# Autodesk Inventor assembly: FE-00004-07
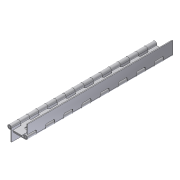
[picture p0: Inventor's stored thumbnail of the model, 180x180]
Saved by Autodesk Inventor 2012 (Build 160160000, 160)
## iProperties
Created: 2008-05-29
Part Number: FE-00004-07
Document SubType Name: Assembly
Designer: narosenberg
Description: Hinge, Stop Plate
Author: narosenberg
## Documents named in this file (4)
- C:\Data Folder\FRC 2012 Field\Components\FE-00004-07.iam
- C:\Data Folder\FRC 2012 Field\Components\FE-00004-07A.ipt
- C:\Data Folder\FRC 2012 Field\Components\FE-00004-07B.ipt
- C:\Data Folder\FRC 2012 Field\Components\FE-00004-07C.ipt
## Components (6 placed, 3 different names)
1. FE-00004-07A:3 — Insert:1, Angle:1, Flush:2
2. FE-00004-07A:2 — Insert:2, Angle:2, Mate:1, Flush:1
3. FE-00004-07B:1 — Insert:1, Insert:4, Angle:1, Mate:1, Flush:1
4. FE-00004-07C:2 — Insert:4
5. FE-00004-07A:1 — Insert:2, Insert:3, Angle:2, Flush:2
6. FE-00004-07C:1 — Insert:3
## Relationships (9: Insert 4, Angle 2, Flush 2, Mate 1)
- Insert:1: FE-00004-07A:3 ↔ FE-00004-07B:1
- Insert:2: FE-00004-07A:2 ↔ FE-00004-07A:1
- Insert:3: FE-00004-07A:1 ↔ FE-00004-07C:1
- Insert:4: FE-00004-07B:1 ↔ FE-00004-07C:2
- Angle:1 (-90 deg): FE-00004-07A:3 ↔ FE-00004-07B:1
- Angle:2 (90 deg): FE-00004-07A:2 ↔ FE-00004-07A:1
- Mate:1: FE-00004-07A:2 ↔ FE-00004-07B:1
- Flush:1: FE-00004-07A:2 ↔ FE-00004-07B:1
- Flush:2 (-44.45 mm): FE-00004-07A:3 ↔ FE-00004-07A:1
